# Autodesk Inventor assembly: N2-vent
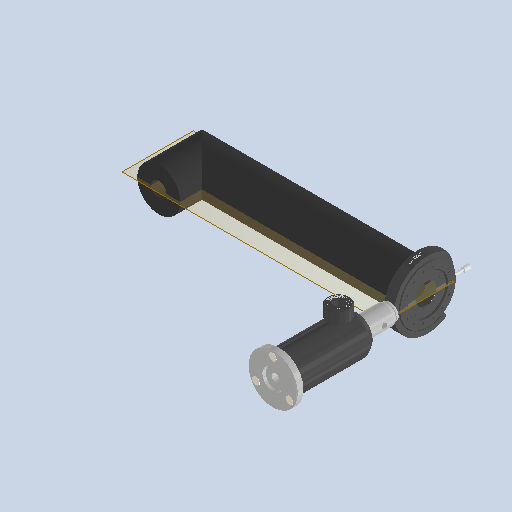
[picture p0: Inventor's stored thumbnail of the model, 512x512]
Saved by Autodesk Inventor 2026.1 (Build 301233000, 233)
## iProperties
Created: 2024-02-07
Part Number: N2-vent
Document SubType Name: Assembly
Designer: Julian
Author: Julian
## Documents named in this file (4)
- C:\Users\user\Desktop\setup_inventor_2025\N2-vent_insulation\N2-vent.iam
- C:\Users\user\Desktop\setup_inventor_2025\N2-vent_insulation\foam tube.ipt
- C:\Users\user\Desktop\setup_inventor_2025\N2-vent_insulation\PH50E_M-Step.ipt
- C:\Users\user\Desktop\setup_inventor_2025\N2-vent_insulation\Iris.ipt
## Components (3 placed, 3 different names)
1. foam tube:1 — Passend:1, Passend:2, Fluchtend:1
2. PH50E_M-Step:1 — Passend:3, Fluchtend:1
3. Iris:1 — Passend:1, Passend:2, Passend:3
## Relationships (4: Mate 3, Flush 1)
- Passend:1 [Mate]: foam tube:1 ↔ Iris:1
- Passend:2 [Mate]: foam tube:1 ↔ Iris:1
- Passend:3 [Mate]: PH50E_M-Step:1 ↔ Iris:1
- Fluchtend:1 [Flush] (-70 mm): foam tube:1 ↔ PH50E_M-Step:1
